# Autodesk Inventor assembly: Assembly_v2
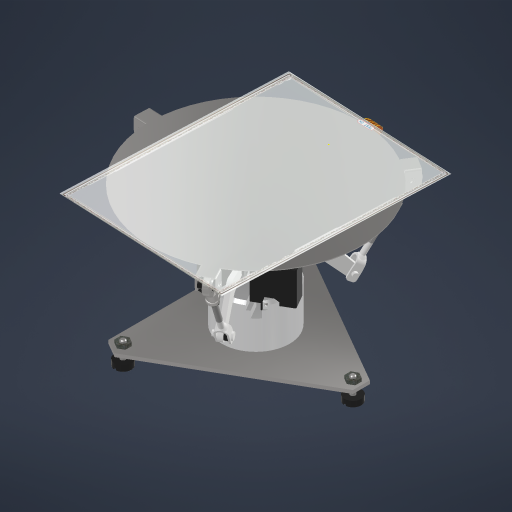
[picture p0: Inventor's stored thumbnail of the model, 512x512]
Saved by Autodesk Inventor 2023 (Build 270158000, 158)
## iProperties
Created: 2023-02-25
Part Number: Assembly_v2
Document SubType Name: Assembly
Designer: roota
Mass: 2505.51 g
Surface Area: 3613.46 cm^2
Volume: 474.073 cm^3
Density: 5.28507 g/cm^3
Author: roota
## Documents named in this file (22)
- D:\GitHub\NTUST-Mechanical-Design\Ball stabilization mechanism\3D CAD files\Mechanical Part CAD files\Assemblies\Assembly_v2.iam
- D:\GitHub\NTUST-Mechanical-Design\Ball stabilization mechanism\3D CAD files\Mechanical Part CAD files\Static Mechanisms\BasePlate.ipt
- D:\GitHub\NTUST-Mechanical-Design\Ball stabilization mechanism\3D CAD files\Mechanical Part CAD files\Static Mechanisms\BaseSupport.ipt
- D:\GitHub\NTUST-Mechanical-Design\Ball stabilization mechanism\3D CAD files\Electrical Hardware CAD files\SERVO\LDX-335MG_Servo_15kg_cm.ipt
- D:\GitHub\NTUST-Mechanical-Design\Ball stabilization mechanism\3D CAD files\Mechanical Part CAD files\Static Mechanisms\ServoCap V2.ipt
- C:\Users\roota\Documents\Inventor\Content Center Files\R2023\en-US\ISO 10642(2)\ISO 10642  - M8  x  80.ipt
- C:\Users\roota\Documents\Inventor\Content Center Files\R2023\en-US\ISO 10642(2)\ISO 10642  - M5  x  12.ipt
- C:\Users\roota\Documents\Inventor\Content Center Files\R2023\en-US\ISO 4762(2)\ISO 4762 - M5 x 12ISO.ipt
- C:\Users\roota\Documents\Inventor\Content Center Files\R2023\en-US\BS EN ISO 4026\BS EN ISO 4168 - M3 x 6(2).ipt
- D:\GitHub\NTUST-Mechanical-Design\Ball stabilization mechanism\3D CAD files\Electrical Hardware CAD files\SERVO\ServoDrive.ipt
- D:\GitHub\NTUST-Mechanical-Design\Ball stabilization mechanism\3D CAD files\Mechanical Part CAD files\Hardware Parts\M6x1 Welded thread fork\M6x1 Welded thread fork.ipt
- D:\GitHub\NTUST-Mechanical-Design\Ball stabilization mechanism\3D CAD files\Mechanical Part CAD files\Hardware Parts\SELF-LUBRIFICATING ROD END\End_6mm.ipt
- D:\GitHub\NTUST-Mechanical-Design\Ball stabilization mechanism\3D CAD files\Mechanical Part CAD files\Hardware Parts\SELF-LUBRIFICATING ROD END\Ball_6mm_male.ipt
- D:\GitHub\NTUST-Mechanical-Design\Ball stabilization mechanism\3D CAD files\Mechanical Part CAD files\Static Mechanisms\rod pin.ipt
- C:\Users\roota\Documents\Inventor\Content Center Files\R2023\en-US\JIS B 2804 E\_JIS B 2804 E - 5 - 6.ipt
- D:\GitHub\NTUST-Mechanical-Design\Ball stabilization mechanism\3D CAD files\Mechanical Part CAD files\Static Mechanisms\4mm spacer.ipt
- D:\GitHub\NTUST-Mechanical-Design\Ball stabilization mechanism\3D CAD files\Mechanical Part CAD files\Static Mechanisms\BalancePlate.ipt
- D:\GitHub\NTUST-Mechanical-Design\Ball stabilization mechanism\3D CAD files\Electrical Hardware CAD files\12_1_INCH_TOUCHSCREEN\12inch Touchscreen.ipt
- C:\Users\roota\Documents\Inventor\Content Center Files\R2023\en-US\ISO 4036(2)\ISO 4036 - M6(2).ipt
- D:\GitHub\NTUST-Mechanical-Design\Ball stabilization mechanism\3D CAD files\Mechanical Part CAD files\Hardware Parts\M6x1 Feet.ipt
- C:\Users\roota\Documents\Inventor\Content Center Files\R2023\en-US\ISO 4036(2)\ISO 4036 - M8(2).ipt
- D:\GitHub\NTUST-Mechanical-Design\Ball stabilization mechanism\3D CAD files\Mechanical Part CAD files\Hardware Parts\LKBK4-L43-S41-Q130-M3-HA6-T5.ipt
## Components (64 placed, 21 different names)
1. BasePlate:1 — Mate:46, Mate:47, Mate:48, Mate:49, Mate:50, Mate:51, Mate:63, Mate:64, Mate:65, Mate:66, Insert:33, Insert:34, Insert:35, Insert:36, Insert:37, Insert:38
2. BaseSupport:1 — Mate:49, Mate:50, Mate:51, Mate:52, Mate:53, Mate:54, Mate:55, Mate:56, Mate:57, Mate:58, Mate:59, Mate:60, Mate:67, Mate:68, Mate:69
3. LDX-335MG_Servo_15kg_cm:1 — Mate:52, Mate:53, Mate:54, Mate:61, Insert:1, Insert:2, Insert:39
4. LDX-335MG_Servo_15kg_cm:2 — Mate:55, Mate:59, Mate:60, Insert:3, Insert:4, Insert:40
5. LDX-335MG_Servo_15kg_cm:3 — Mate:56, Mate:57, Mate:58, Insert:5, Insert:6, Insert:41
6. ServoCap V2:1 — Mate:61, Mate:62, Mate:70, Mate:82
7. DIN EN ISO 10642 M8  x  80:1 — Mate:62
8. DIN EN ISO 10642 M5  x  12:1 — Mate:63
9. DIN EN ISO 10642 M5  x  12:2 — Mate:64
10. DIN EN ISO 10642 M5  x  12:3 — Mate:65
11. DIN EN ISO 10642 M5  x  12:4 — Mate:66
12. ISO 4762 M5 x 12:1 — Insert:1
13. ISO 4762 M5 x 12:2 — Insert:2
14. ISO 4762 M5 x 12:3 — Insert:3
15. ISO 4762 M5 x 12:4 — Insert:4, Mate:70
16. ISO 4762 M5 x 12:5 — Insert:5
17. ISO 4762 M5 x 12:6 — Insert:6
18. BS EN ISO 4026 - Metric M3 x 6:1 — Mate:67
19. BS EN ISO 4026 - Metric M3 x 6:2 — Mate:68
20. BS EN ISO 4026 - Metric M3 x 6:3 — Mate:69
21. M6x1 Welded thread fork:1 — Insert:16, Angle:1, Insert:42, Mate:96
22. M6x1 Welded thread fork:2 — Insert:18, Angle:2, Mate:84, Insert:43, Mate:95
23. M6x1 Welded thread fork:3 — Insert:17, Angle:3, Mate:89, Mate:90, Mate:94
24. End_6mm:1 — Insert:16, Angle:1, Tangent:3, Insert:32
25. End_6mm:2 — Insert:17, Angle:3, Tangent:1, Insert:31
26. End_6mm:3 — Insert:18, Angle:2, Tangent:2, Mate:85
27. Ball_6mm_male:1 — Tangent:1, Insert:25, Insert:26
28. Ball_6mm_male:2 — Tangent:2, Insert:29, Insert:30
29. Ball_6mm_male:3 — Tangent:3, Insert:27, Insert:28
30. rod pin:1 — Insert:23, Insert:24, Mate:71, Mate:74
31. rod pin:2 — Insert:19, Insert:20, Mate:72
32. rod pin:3 — Insert:21, Insert:22, Mate:73
33. JIS B 2804 E 5:1 — Insert:19
34. JIS B 2804 E 5:2 — Insert:20, Mate:78
35. JIS B 2804 E 5:3 — Insert:21, Mate:81
36. JIS B 2804 E 5:4 — Insert:22
37. JIS B 2804 E 5:5 — Insert:23
38. JIS B 2804 E 5:6 — Insert:24
39. 4mm spacer:1 — Insert:25, Mate:71, Mate:75
40. 4mm spacer:2 — Insert:26
41. 4mm spacer:3 — Insert:27, Mate:73, Mate:79
42. 4mm spacer:4 — Insert:28, Mate:80
43. 4mm spacer:5 — Insert:29, Mate:76, Mate:77
44. 4mm spacer:6 — Insert:30, Mate:72
45. BalancePlate:1 — Mate:74, Mate:75, Mate:76, Mate:77, Mate:78, Mate:79, Mate:80, Mate:81, Mate:82, Mate:83, Flush:1, Flush:2
46. 12inch Touchscreen:1 — Mate:83, Flush:1, Flush:2
47. ISO 4036 M6:1 — Insert:31
48. ISO 4036 M6:2 — Mate:84, Mate:85
49. ISO 4036 M6:3 — Insert:32
50. M6x1 Feet:1 — Insert:33
51. M6x1 Feet:2 — Insert:34
52. M6x1 Feet:3 — Insert:35
53. ISO 4036 M8:1 — Insert:36
54. ISO 4036 M8:2 — Insert:37
55. ISO 4036 M8:3 — Insert:38
56. ServoDrive:1 — Insert:39, Insert:46, Mate:93
57. ServoDrive:2 — Insert:40, Insert:48, Mate:91
58. ServoDrive:3 — Insert:41, Insert:47, Mate:92
59. 4mm spacer:7 — Mate:88, Mate:89, Mate:90
60. 4mm spacer:8 — Insert:42, Mate:86
61. 4mm spacer:9 — Insert:43, Mate:87
62. LKBK4-L43-S41-Q130-M3-HA6-T5:3 — Insert:46, Mate:88, Mate:93, Mate:94
63. LKBK4-L43-S41-Q130-M3-HA6-T5:4 — Insert:47, Mate:87, Mate:92, Mate:95
64. LKBK4-L43-S41-Q130-M3-HA6-T5:5 — Insert:48, Mate:86, Mate:91, Mate:96
## Relationships (96: Mate 51, Insert 37, Angle 3, Tangent 3, Flush 2)
- Mate:46: BasePlate:1
- Mate:47: BasePlate:1
- Mate:48: BasePlate:1
- Mate:49: BasePlate:1 ↔ BaseSupport:1
- Mate:50: BasePlate:1 ↔ BaseSupport:1
- Mate:51: BasePlate:1 ↔ BaseSupport:1
- Mate:52: BaseSupport:1 ↔ LDX-335MG_Servo_15kg_cm:1
- Mate:53: BaseSupport:1 ↔ LDX-335MG_Servo_15kg_cm:1
- Mate:54: BaseSupport:1 ↔ LDX-335MG_Servo_15kg_cm:1
- Mate:55: BaseSupport:1 ↔ LDX-335MG_Servo_15kg_cm:2
- Mate:56: BaseSupport:1 ↔ LDX-335MG_Servo_15kg_cm:3
- Mate:57: BaseSupport:1 ↔ LDX-335MG_Servo_15kg_cm:3
- Mate:58: BaseSupport:1 ↔ LDX-335MG_Servo_15kg_cm:3
- Mate:59: BaseSupport:1 ↔ LDX-335MG_Servo_15kg_cm:2
- Mate:60: BaseSupport:1 ↔ LDX-335MG_Servo_15kg_cm:2
- Mate:61: LDX-335MG_Servo_15kg_cm:1 ↔ ServoCap V2:1
- Mate:62: ServoCap V2:1 ↔ DIN EN ISO 10642 M8  x  80:1
- Mate:63: BasePlate:1 ↔ DIN EN ISO 10642 M5  x  12:1
- Mate:64: BasePlate:1 ↔ DIN EN ISO 10642 M5  x  12:2
- Mate:65: BasePlate:1 ↔ DIN EN ISO 10642 M5  x  12:3
- Mate:66: BasePlate:1 ↔ DIN EN ISO 10642 M5  x  12:4
- Insert:1: LDX-335MG_Servo_15kg_cm:1 ↔ ISO 4762 M5 x 12:1
- Insert:2: LDX-335MG_Servo_15kg_cm:1 ↔ ISO 4762 M5 x 12:2
- Insert:3: LDX-335MG_Servo_15kg_cm:2 ↔ ISO 4762 M5 x 12:3
- Insert:4: LDX-335MG_Servo_15kg_cm:2 ↔ ISO 4762 M5 x 12:4
- Insert:5: LDX-335MG_Servo_15kg_cm:3 ↔ ISO 4762 M5 x 12:5
- Insert:6: LDX-335MG_Servo_15kg_cm:3 ↔ ISO 4762 M5 x 12:6
- Mate:67: BaseSupport:1 ↔ BS EN ISO 4026 - Metric M3 x 6:1
- Mate:68: BaseSupport:1 ↔ BS EN ISO 4026 - Metric M3 x 6:2
- Mate:69: BaseSupport:1 ↔ BS EN ISO 4026 - Metric M3 x 6:3
- Mate:70: ServoCap V2:1 ↔ ISO 4762 M5 x 12:4
- Insert:16 (-8 mm): M6x1 Welded thread fork:1 ↔ End_6mm:1
- Insert:17 (-8 mm): M6x1 Welded thread fork:3 ↔ End_6mm:2
- Insert:18 (-8 mm): M6x1 Welded thread fork:2 ↔ End_6mm:3
- Angle:1 (0 deg): M6x1 Welded thread fork:1 ↔ End_6mm:1
- Angle:2 (0 deg): M6x1 Welded thread fork:2 ↔ End_6mm:3
- Angle:3 (0 deg): M6x1 Welded thread fork:3 ↔ End_6mm:2
- Tangent:1: End_6mm:2 ↔ Ball_6mm_male:1
- Tangent:2: End_6mm:3 ↔ Ball_6mm_male:2
- Tangent:3: End_6mm:1 ↔ Ball_6mm_male:3
- Insert:19: rod pin:2 ↔ JIS B 2804 E 5:1
- Insert:20: rod pin:2 ↔ JIS B 2804 E 5:2
- Insert:21: rod pin:3 ↔ JIS B 2804 E 5:3
- Insert:22: rod pin:3 ↔ JIS B 2804 E 5:4
- Insert:23: rod pin:1 ↔ JIS B 2804 E 5:5
- Insert:24: rod pin:1 ↔ JIS B 2804 E 5:6
- Insert:25: Ball_6mm_male:1 ↔ 4mm spacer:1
- Insert:26: Ball_6mm_male:1 ↔ 4mm spacer:2
- Insert:27: Ball_6mm_male:3 ↔ 4mm spacer:3
- Insert:28: Ball_6mm_male:3 ↔ 4mm spacer:4
- Insert:29: Ball_6mm_male:2 ↔ 4mm spacer:5
- Insert:30: Ball_6mm_male:2 ↔ 4mm spacer:6
- Mate:71: rod pin:1 ↔ 4mm spacer:1
- Mate:72: rod pin:2 ↔ 4mm spacer:6
- Mate:73: rod pin:3 ↔ 4mm spacer:3
- Mate:74: rod pin:1 ↔ BalancePlate:1
- Mate:75: 4mm spacer:1 ↔ BalancePlate:1
- Mate:76: 4mm spacer:5 ↔ BalancePlate:1
- Mate:77: 4mm spacer:5 ↔ BalancePlate:1
- Mate:78: JIS B 2804 E 5:2 ↔ BalancePlate:1
- Mate:79: 4mm spacer:3 ↔ BalancePlate:1
- Mate:80: 4mm spacer:4 ↔ BalancePlate:1
- Mate:81: JIS B 2804 E 5:3 ↔ BalancePlate:1
- Mate:82 (60 mm): ServoCap V2:1 ↔ BalancePlate:1
- Mate:83: BalancePlate:1 ↔ 12inch Touchscreen:1
- Flush:1 (40 mm): BalancePlate:1 ↔ 12inch Touchscreen:1
- Flush:2 (-120 mm): BalancePlate:1 ↔ 12inch Touchscreen:1
- Insert:31: End_6mm:2 ↔ ISO 4036 M6:1
- Mate:84: M6x1 Welded thread fork:2 ↔ ISO 4036 M6:2
- Mate:85: End_6mm:3 ↔ ISO 4036 M6:2
- Insert:32: End_6mm:1 ↔ ISO 4036 M6:3
- Insert:33 (-10 mm): BasePlate:1 ↔ M6x1 Feet:1
- Insert:34 (-10 mm): BasePlate:1 ↔ M6x1 Feet:2
- Insert:35 (-10 mm): BasePlate:1 ↔ M6x1 Feet:3
- Insert:36: BasePlate:1 ↔ ISO 4036 M8:1
- Insert:37: BasePlate:1 ↔ ISO 4036 M8:2
- Insert:38: BasePlate:1 ↔ ISO 4036 M8:3
- Insert:39: LDX-335MG_Servo_15kg_cm:1 ↔ ServoDrive:1
- Insert:40: LDX-335MG_Servo_15kg_cm:2 ↔ ServoDrive:2
- Insert:41: LDX-335MG_Servo_15kg_cm:3 ↔ ServoDrive:3
- Insert:42: M6x1 Welded thread fork:1 ↔ 4mm spacer:8
- Insert:43: M6x1 Welded thread fork:2 ↔ 4mm spacer:9
- Insert:46: ServoDrive:1 ↔ LKBK4-L43-S41-Q130-M3-HA6-T5:3
- Insert:47: ServoDrive:3 ↔ LKBK4-L43-S41-Q130-M3-HA6-T5:4
- Insert:48: ServoDrive:2 ↔ LKBK4-L43-S41-Q130-M3-HA6-T5:5
- Mate:86: 4mm spacer:8 ↔ LKBK4-L43-S41-Q130-M3-HA6-T5:5
- Mate:87: 4mm spacer:9 ↔ LKBK4-L43-S41-Q130-M3-HA6-T5:4
- Mate:88: 4mm spacer:7 ↔ LKBK4-L43-S41-Q130-M3-HA6-T5:3
- Mate:89: M6x1 Welded thread fork:3 ↔ 4mm spacer:7
- Mate:90: M6x1 Welded thread fork:3 ↔ 4mm spacer:7
- Mate:91: ServoDrive:2 ↔ LKBK4-L43-S41-Q130-M3-HA6-T5:5
- Mate:92: ServoDrive:3 ↔ LKBK4-L43-S41-Q130-M3-HA6-T5:4
- Mate:93: ServoDrive:1 ↔ LKBK4-L43-S41-Q130-M3-HA6-T5:3
- Mate:94: M6x1 Welded thread fork:3 ↔ LKBK4-L43-S41-Q130-M3-HA6-T5:3
- Mate:95: M6x1 Welded thread fork:2 ↔ LKBK4-L43-S41-Q130-M3-HA6-T5:4
- Mate:96: M6x1 Welded thread fork:1 ↔ LKBK4-L43-S41-Q130-M3-HA6-T5:5
## Named parameters: AngleX = 5 deg, AngleY = 5 deg
